# Autodesk Inventor assembly: Bird_wing_assembly_V1
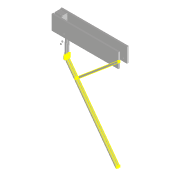
[picture p0: Inventor's stored thumbnail of the model, 180x180]
Saved by Autodesk Inventor 2022 (Build 260153000, 153)
## iProperties
Created: 2022-07-06
Part Number: Bird_wing_assembly_V1
Document SubType Name: Assembly
Designer: dell
Author: dell
## Documents named in this file (11)
- D:\xxxx\Uni\Part IV\MECHENG_700\Part_IV_project_CAD\Bird_skeleton_prototypes\Wing_drone_V1\Bird_wing_V1\Bird_wing_assembly_V1.iam
- D:\xxxx\Uni\Part IV\MECHENG_700\Part_IV_project_CAD\Bird_skeleton_prototypes\Wing_drone_V1\Bird_wing_V1\Wing_base.ipt
- D:\xxxx\Uni\Part IV\MECHENG_700\Part_IV_project_CAD\Bird_skeleton_prototypes\Wing_drone_V1\Bird_wing_V1\Motor_adaptor.ipt
- D:\xxxx\Uni\Part IV\MECHENG_700\Part_IV_project_CAD\Bird_skeleton_prototypes\Wing_drone_V1\Bird_wing_V1\Wing_arm_1.ipt
- D:\xxxx\Uni\Part IV\MECHENG_700\Part_IV_project_CAD\Bird_skeleton_prototypes\Wing_drone_V1\Bird_wing_V1\Wing_joint_link.ipt
- D:\xxxx\Uni\Part IV\MECHENG_700\Part_IV_project_CAD\Bird_skeleton_prototypes\Wing_drone_V1\Bird_wing_V1\Wing_arm_2.ipt
- D:\xxxx\Uni\Part IV\MECHENG_700\Part_IV_project_CAD\Bird_skeleton_prototypes\Wing_drone_V1\Bird_wing_V1\Wing_arm_3.ipt
- D:\xxxx\Uni\Part IV\MECHENG_700\Part_IV_project_CAD\Bird_skeleton_prototypes\Wing_drone_V1\Bird_wing_V1\57545K764_Metal Worm Gear.ipt
- D:\xxxx\Uni\Part IV\MECHENG_700\Part_IV_project_CAD\Bird_skeleton_prototypes\Wing_drone_V1\Bird_wing_V1\Motor_assembly.iam
- D:\xxxx\Uni\Part IV\MECHENG_700\Part_IV_project_CAD\Bird_skeleton_prototypes\Wing_drone_V1\Bird_wing_V1\M3_washer.ipt
- D:\xxxx\Uni\Part IV\MECHENG_700\Part_IV_project_CAD\Bird_skeleton_prototypes\Wing_drone_V1\Bird_wing_V1\Bearing_4_7_2.5mm.ipt
## Components (18 placed, 10 different names)
1. Motor_adaptor:1 — Mate:10, Mate:12, Mate:14, Mate:15, Mate:39, Mate:40
2. Wing_arm_1:1 — Mate:10, Mate:12, Mate:16, Mate:17, Flush:1, Mate:26, Mate:27, Flush:4, Mate:40, Mate:41, Mate:45, Mate:47, Mate:48
3. Wing_arm_1:2 — Mate:14, Mate:15, Mate:24, Mate:25, Flush:3, Mate:33, Mate:34, Mate:38, Mate:39
4. Wing_joint_link:1 — Mate:24, Mate:25, Flush:3
5. Wing_joint_link:2 — Mate:16, Mate:17, Flush:1, Mate:19, Mate:20, Mate:22, Mate:23
6. Wing_joint_link:3 — Mate:26, Mate:27, Flush:4
7. Wing_arm_2:1 — Mate:19, Mate:20, Flush:2, Mate:28, Mate:29
8. Wing_arm_2:2 — Mate:22, Mate:23, Flush:2
9. Wing_arm_3:1 — Mate:28, Mate:29, Mate:37
10. 57545K764_Metal Worm Gear:1 — Mate:33, Mate:34, Mate:38
11. Motor_assembly:5 [sub-assembly]
12. Wing_base:1 — Mate:37, Mate:41, Mate:42, Mate:43
13. M3_washer:1 — Mate:42, Mate:43, Mate:44, Mate:48
14. Bearing_4_7_2.5mm:1 — Mate:44, Mate:45, Mate:46
15. Bearing_4_7_2.5mm:2 — Mate:46, Mate:47
16. Bearing_4_7_2.5mm:3
17. Bearing_4_7_2.5mm:4
18. Wing_base:2
## Relationships (34: Mate 30, Flush 4)
- Mate:10: Motor_adaptor:1 ↔ Wing_arm_1:1
- Mate:12: Motor_adaptor:1 ↔ Wing_arm_1:1
- Mate:14: Motor_adaptor:1 ↔ Wing_arm_1:2
- Mate:15: Motor_adaptor:1 ↔ Wing_arm_1:2
- Mate:16: Wing_arm_1:1 ↔ Wing_joint_link:2
- Mate:17: Wing_arm_1:1 ↔ Wing_joint_link:2
- Flush:1: Wing_arm_1:1 ↔ Wing_joint_link:2
- Mate:19: Wing_joint_link:2 ↔ Wing_arm_2:1
- Mate:20: Wing_joint_link:2 ↔ Wing_arm_2:1
- Mate:22: Wing_joint_link:2 ↔ Wing_arm_2:2
- Mate:23: Wing_joint_link:2 ↔ Wing_arm_2:2
- Flush:2: Wing_arm_2:1 ↔ Wing_arm_2:2
- Mate:24: Wing_arm_1:2 ↔ Wing_joint_link:1
- Mate:25: Wing_arm_1:2 ↔ Wing_joint_link:1
- Flush:3: Wing_arm_1:2 ↔ Wing_joint_link:1
- Mate:26: Wing_arm_1:1 ↔ Wing_joint_link:3
- Mate:27: Wing_arm_1:1 ↔ Wing_joint_link:3
- Flush:4: Wing_arm_1:1 ↔ Wing_joint_link:3
- Mate:28: Wing_arm_2:1 ↔ Wing_arm_3:1
- Mate:29: Wing_arm_2:1 ↔ Wing_arm_3:1
- Mate:33: Wing_arm_1:2 ↔ 57545K764_Metal Worm Gear:1
- Mate:34: Wing_arm_1:2 ↔ 57545K764_Metal Worm Gear:1
- Mate:37: Wing_arm_3:1 ↔ Wing_base:1
- Mate:38: Wing_arm_1:2 ↔ 57545K764_Metal Worm Gear:1
- Mate:39: Motor_adaptor:1 ↔ Wing_arm_1:2
- Mate:40: Motor_adaptor:1 ↔ Wing_arm_1:1
- Mate:41: Wing_arm_1:1 ↔ Wing_base:1
- Mate:42: Wing_base:1 ↔ M3_washer:1
- Mate:43: Wing_base:1 ↔ M3_washer:1
- Mate:44: M3_washer:1 ↔ Bearing_4_7_2.5mm:1
- Mate:45: Wing_arm_1:1 ↔ Bearing_4_7_2.5mm:1
- Mate:46: Bearing_4_7_2.5mm:1 ↔ Bearing_4_7_2.5mm:2
- Mate:47: Wing_arm_1:1 ↔ Bearing_4_7_2.5mm:2
- Mate:48: Wing_arm_1:1 ↔ M3_washer:1
